# Autodesk Inventor assembly: m4 bearing assembly
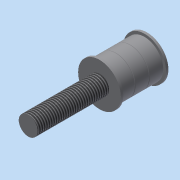
[picture p0: Inventor's stored thumbnail of the model, 180x180]
Saved by Autodesk Inventor 2015 (Build 190159000, 159)
## iProperties
Created: 2016-09-08
Part Number: m4 bearing assembly
Document SubType Name: Assembly
Designer: Dustin
Author: Dustin
## Documents named in this file (4)
- E:\Documents\3D Printer\LetzteBot3DPrinter\Inventor Files\IAM Files\M4BA1.iam
- E:\Documents\3D Printer\LetzteBot3DPrinter\Inventor Files\IPT Files\S440.ipt
- E:\Documents\3D Printer\LetzteBot3DPrinter\Inventor Files\IPT Files\LR84ZZ.ipt
- E:\Documents\3D Printer\LetzteBot3DPrinter\Inventor Files\IPT Files\W4.ipt
## Components (6 placed, 3 different names)
1. S440:1 — Angle:1, Tangent:1, Mate:1, Angle:2, Tangent:2, Angle:3, Tangent:3, Insert:1
2. LR84ZZ:1 — Angle:3, Tangent:3, Mate:3, Insert:2
3. LR84ZZ:2 — Angle:2, Tangent:2, Mate:2, Mate:3
4. LR84ZZ:3 — Angle:1, Tangent:1, Mate:1, Mate:2
5. W4:1 — Insert:1
6. W4:2 — Insert:2
## Relationships (11: Angle 3, Tangent 3, Mate 3, Insert 2)
- Angle:1 (0 deg): S440:1 ↔ LR84ZZ:3
- Tangent:1: S440:1 ↔ LR84ZZ:3
- Mate:1 (0.5 mm): S440:1 ↔ LR84ZZ:3
- Angle:2 (0 deg): S440:1 ↔ LR84ZZ:2
- Tangent:2: S440:1 ↔ LR84ZZ:2
- Mate:2: LR84ZZ:2 ↔ LR84ZZ:3
- Angle:3 (0 deg): S440:1 ↔ LR84ZZ:1
- Tangent:3: S440:1 ↔ LR84ZZ:1
- Mate:3: LR84ZZ:1 ↔ LR84ZZ:2
- Insert:1: S440:1 ↔ W4:1
- Insert:2: LR84ZZ:1 ↔ W4:2
